# Autodesk Inventor assembly: WCP Polycord Pulley Assembled States
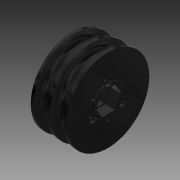
[picture p0: Inventor's stored thumbnail of the model, 180x180]
Saved by Autodesk Inventor 2022 (Build 260153000, 153)
## iProperties
Created: 2021-12-28
Part Number: WCP Polycord Pulley Assembled States
Document SubType Name: Assembly
## iProperties of the stored document MemberDocs/x0elbbrcpJs2a0dip5zlvg5xyFh
Created: 2021-12-28
Part Number: WCP Polycord Pulley Assembled States
Document SubType Name: Assembly
## Documents named in this file (2)
- C:\Users\Cal\Desktop\Robotics\Design\Collaborative\Collaborative Parts Library\Power Transfer\Belts and Pullies\WCP Polycord Pulley Assembled States.iam
- C:\Users\Cal\Desktop\Robotics\Design\Collaborative\Collaborative Parts Library\Power Transfer\Belts and Pullies\WCP Polycord Pulley States.ipt
## Components (3 placed, 1 different names)
1. WCP Polycord Pulley States:1 — Mate:1, Flush:1, Mate:2, Flush:2, Symmetry:1, Mate:5, Mate:6
2. WCP Polycord Pulley States:2 — Mate:1, Flush:1, Symmetry:1, Mate:5
3. WCP Polycord Pulley States:3 — Mate:3, Mate:4, Mate:6
## Component patterns: (1 elements, first: WCP Polycord Pulley States:3)
## Relationships (9: Mate 6, Flush 2, Symmetry 1)
- Mate:1: WCP Polycord Pulley States:1 ↔ WCP Polycord Pulley States:2
- Flush:1: WCP Polycord Pulley States:1 ↔ WCP Polycord Pulley States:2
- Mate:2: WCP Polycord Pulley States:1
- Flush:2: WCP Polycord Pulley States:1
- Symmetry:1: WCP Polycord Pulley States:1 ↔ WCP Polycord Pulley States:2
- Mate:3: WCP Polycord Pulley States:3
- Mate:4: WCP Polycord Pulley States:3
- Mate:5 (9.3853 mm): WCP Polycord Pulley States:1 ↔ WCP Polycord Pulley States:2
- Mate:6: WCP Polycord Pulley States:1 ↔ WCP Polycord Pulley States:3
## Named parameters: PatternWidth = 9.3853 mm, PulleyCount = 2
